# Autodesk Inventor assembly: 30mm Fan
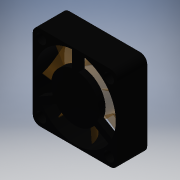
[picture p0: Inventor's stored thumbnail of the model, 180x180]
Saved by Autodesk Inventor 2016 SP1 (Build 200210100, 210)
## iProperties
Created: 2015-12-17
Part Number: 30mm Fan
Document SubType Name: Assembly
Designer: roduino
Title: /vol/tmp/translate-1970156840469106288/56733729e4b0e545db4b6a25.step
## Documents named in this file (3)
- E:\GitHub\kossel-XXL\30mm Fan.iam
- E:\GitHub\kossel-XXL\Part 1.ipt
- E:\GitHub\kossel-XXL\Part 2.ipt
## Components (2 placed, 2 different names)
1. Part 1 — Mate:1, Mate:2
2. Part 2 — Mate:1, Mate:2
## Relationships (2: Mate 2)
- Mate:1: Part 1 ↔ Part 2
- Mate:2: Part 1 ↔ Part 2
